# Autodesk Inventor assembly: VENTILO 5SPI
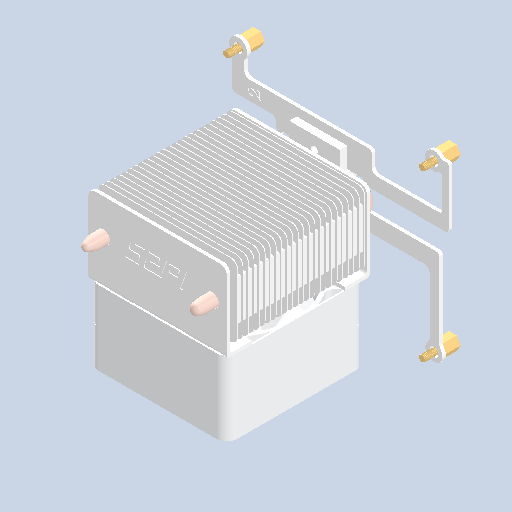
[picture p0: Inventor's stored thumbnail of the model, 512x512]
Saved by Autodesk Inventor 2024 (Build 280153000, 153)
## iProperties
Created: 2022-12-04
Part Number: VENTILO 5SPI
Document SubType Name: Assembly
Designer: 18179
Sending System: Autodesk Translation Framework v11.17.0.187
Preprocessor: ST-DEVELOPER v19.2
Title: VENTILO 5SPI.step
## Documents named in this file (3)
- C:\Users\18179\Desktop\TuppyMkIV_GitHub\TuppyMkIV\CAD\IceTower.iam
- C:\Users\18179\Desktop\TuppyMkIV_GitHub\TuppyMkIV\CAD\VENTILO 5SPI\FAN.ipt
- C:\Users\18179\Desktop\TuppyMkIV_GitHub\TuppyMkIV\CAD\VENTILO 5SPI\Part9.ipt
## Components (3 placed, 2 different names)
1. FAN:1 — Flush:1, Flush:2, Mate:1
2. Part9
3. FAN:2 — Flush:1, Flush:2, Mate:1
## Relationships (3: Flush 2, Mate 1)
- Flush:1: FAN:1 ↔ FAN:2
- Flush:2: FAN:1 ↔ FAN:2
- Mate:1: FAN:1 ↔ FAN:2
